# Autodesk Inventor assembly: Extrusora ensamblaje
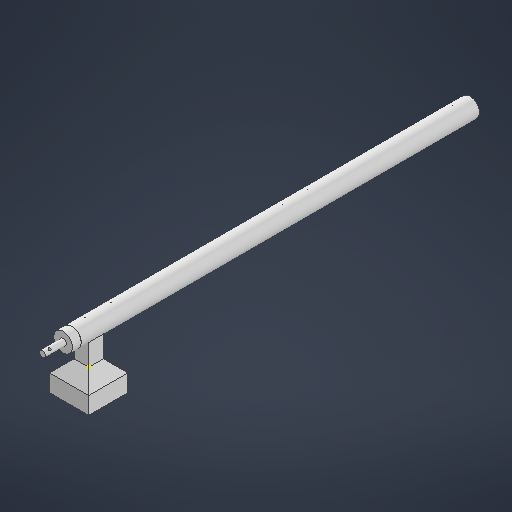
[picture p0: Inventor's stored thumbnail of the model, 512x512]
Saved by Autodesk Inventor 2026.1 (Build 301233020, 233B)
## iProperties
Created: 2025-12-03
Part Number: Extrusora ensamblaje
Document SubType Name: Assembly
Designer: benja
Author: benja
## Documents named in this file (7)
- C:\Users\benja\OneDrive\Escritorio\extrusora\Extrusora ensamblaje .iam
- C:\Users\benja\OneDrive\Escritorio\extrusora\alimentaciion tornillo .ipt
- C:\Users\benja\OneDrive\Escritorio\extrusora\compresion tornillo.ipt
- C:\Users\benja\OneDrive\Escritorio\extrusora\dosificacion tornillo.ipt
- C:\Users\benja\OneDrive\Escritorio\extrusora\tolva completa.iam
- C:\Users\benja\OneDrive\Escritorio\extrusora\tapa seccion alimentacion.ipt
- C:\Users\benja\OneDrive\Escritorio\extrusora\6201-c-2z.ipt
## Components (6 placed, 6 different names)
1. alimentaciion tornillo :1 — Coincidencia:1, Coincidencia:2, Coincidencia:3, Rotación:2, Coincidencia:7, Rotación:3, Coincidencia:9, Nivelación:1
2. compresion tornillo:1 — Coincidencia:1, Coincidencia:2, Coincidencia:3, Coincidencia:4, Coincidencia:5, Coincidencia:6, Rotación:1, Rotación:2
3. dosificacion tornillo:1 — Coincidencia:4, Coincidencia:5, Coincidencia:6, Rotación:1, Rotación:3
4. tolva completa:1 [sub-assembly] — Coincidencia:7, Nivelación:1, Coincidencia:10
5. tapa seccion alimentacion:1 — Coincidencia:8, Tangente:1, Coincidencia:9, Coincidencia:10
6. 6201-c-2z:1 — Coincidencia:8, Tangente:1
## Relationships (15: Mate 10, RelateRotation 3, Tangent 1, Flush 1)
- Coincidencia:1 [Mate]: alimentaciion tornillo :1 ↔ compresion tornillo:1
- Coincidencia:2 [Mate]: alimentaciion tornillo :1 ↔ compresion tornillo:1
- Coincidencia:3 [Mate]: alimentaciion tornillo :1 ↔ compresion tornillo:1
- Coincidencia:4 [Mate]: compresion tornillo:1 ↔ dosificacion tornillo:1
- Coincidencia:5 [Mate]: compresion tornillo:1 ↔ dosificacion tornillo:1
- Coincidencia:6 [Mate]: compresion tornillo:1 ↔ dosificacion tornillo:1
- Rotación:1 [RelateRotation] (1 ul): compresion tornillo:1 ↔ dosificacion tornillo:1
- Rotación:2 [RelateRotation] (1.356 ul): alimentaciion tornillo :1 ↔ compresion tornillo:1
- Coincidencia:7 [Mate]: alimentaciion tornillo :1 ↔ tolva completa:1
- Rotación:3 [RelateRotation] (0.914 ul): alimentaciion tornillo :1 ↔ dosificacion tornillo:1
- Coincidencia:8 [Mate]: tapa seccion alimentacion:1 ↔ 6201-c-2z:1
- Tangente:1: tapa seccion alimentacion:1 ↔ 6201-c-2z:1
- Coincidencia:9 [Mate]: alimentaciion tornillo :1 ↔ tapa seccion alimentacion:1
- Nivelación:1 [Flush]: alimentaciion tornillo :1 ↔ tolva completa:1
- Coincidencia:10 [Mate]: tolva completa:1 ↔ tapa seccion alimentacion:1
